# Autodesk Inventor assembly: roller
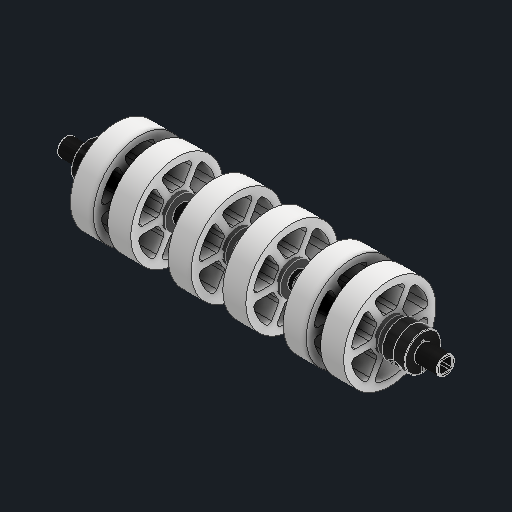
[picture p0: Inventor's stored thumbnail of the model, 512x512]
Saved by Autodesk Inventor 2024 (Build 280153000, 153)
## iProperties
Created: 2024-02-24
Part Number: roller
Document SubType Name: Assembly
Designer: Averey Ku
Author: Averey Ku
## Documents named in this file (8)
- D:\vex_robotics\hardware\cad\smolbot\intake\roller.iam
- D:\vex_robotics\hardware\cad\VEX-CAD-Inventor-1.41\Motion\Wheels\Flex Wheels\2.000 Flex Wheel\2.000 30A .500.ipt
- D:\vex_robotics\hardware\cad\VEX-CAD-Inventor-1.41\Motion\Wheels\Flex Wheels\VersaHex Adapters .125.ipt
- D:\vex_robotics\hardware\cad\VEX-CAD-Inventor-1.41\Motion\Shaft HS\HS Spacer\HSpacer .1250.ipt
- D:\vex_robotics\hardware\cad\VEX-CAD-Inventor-1.41\Motion\Shaft HS\HS Spacer\HSpacer .5000.ipt
- D:\vex_robotics\hardware\cad\VEX-CAD-Inventor-1.41\Motion\Shaft HS\HS Shaft Collar.ipt
- D:\vex_robotics\hardware\cad\VEX-CAD-Inventor-1.41\Motion\Wheels\Flex Wheels\2.000 Flex Wheel.ipt
- D:\vex_robotics\hardware\cad\VEX-CAD-Inventor-1.41\Motion\Shaft HS\HS Spacer.ipt
## Components (31 placed, 5 different names)
1. 2.000 30A .500:2 — Insert:20
2. VersaHex Adapters .125:3
3. VersaHex Adapters .125:4 — Insert:18, Insert:20
4. 2.000 30A .500:3 — Insert:21, Insert:22
5. VersaHex Adapters .125:5 — Insert:19, Insert:21
6. VersaHex Adapters .125:6 — Insert:22
7. 2.000 30A .500:4 — Insert:35
8. VersaHex Adapters .125:7 — Insert:23
9. VersaHex Adapters .125:8 — Insert:35, Insert:36
10. 2.000 30A .500:5 — Insert:33, Insert:34
11. VersaHex Adapters .125:9 — Insert:34
12. VersaHex Adapters .125:10 — Insert:31, Insert:33
13. 2.000 30A .500:6 — Insert:26, Insert:28
14. VersaHex Adapters .125:11 — Insert:28
15. VersaHex Adapters .125:12 — Insert:25, Insert:26
16. 2.000 30A .500:7 — Insert:27, Insert:30
17. VersaHex Adapters .125:13 — Insert:24, Insert:27, Insert:29
18. VersaHex Adapters .125:14 — Insert:30, Insert:32
19. HSpacer .5000:3 — Insert:36
20. HS Shaft Collar:1 — Insert:38
21. HSpacer .1250:6
22. HS Shaft Collar:2 — Insert:37
23. HSpacer .1250:7 — Insert:32
24. HSpacer .5000:8
25. HSpacer .1250:9 — Insert:31
26. HSpacer .5000:10
27. HSpacer .1250:11 — Insert:23
28. HSpacer .1250:14 — Insert:18, Insert:19
29. HSpacer .1250:15 — Insert:24, Insert:25, Insert:29
30. HSpacer .5000:16 — Insert:37
31. HSpacer .5000:17 — Insert:38
## Relationships (29: Insert 29)
- [Insert]: VersaHex Adapters .125:9 ↔ HSpacer .5000:3
- [Insert]: HS Shaft Collar:1 ↔ HSpacer .1250:6
- [Insert]: VersaHex Adapters .125:3 ↔ HSpacer .1250:6
- [Insert]: HS Shaft Collar:2 ↔ HSpacer .1250:7
- [Insert]: HSpacer .5000:8 ↔ HSpacer .1250:9
- [Insert]: HSpacer .5000:10 ↔ HSpacer .1250:11
- [Insert]: VersaHex Adapters .125:6 ↔ HSpacer .5000:10
- [Insert]: VersaHex Adapters .125:11 ↔ HSpacer .5000:8
- Insert:18: VersaHex Adapters .125:4 ↔ HSpacer .1250:14
- Insert:19: VersaHex Adapters .125:5 ↔ HSpacer .1250:14
- Insert:20: 2.000 30A .500:2 ↔ VersaHex Adapters .125:4
- Insert:21: 2.000 30A .500:3 ↔ VersaHex Adapters .125:5
- Insert:22: 2.000 30A .500:3 ↔ VersaHex Adapters .125:6
- Insert:23: VersaHex Adapters .125:7 ↔ HSpacer .1250:11
- Insert:24: VersaHex Adapters .125:13 ↔ HSpacer .1250:15
- Insert:25: VersaHex Adapters .125:12 ↔ HSpacer .1250:15
- Insert:26: 2.000 30A .500:6 ↔ VersaHex Adapters .125:12
- Insert:27: 2.000 30A .500:7 ↔ VersaHex Adapters .125:13
- Insert:28: 2.000 30A .500:6 ↔ VersaHex Adapters .125:11
- Insert:29: VersaHex Adapters .125:13 ↔ HSpacer .1250:15
- Insert:30: 2.000 30A .500:7 ↔ VersaHex Adapters .125:14
- Insert:31: VersaHex Adapters .125:10 ↔ HSpacer .1250:9
- Insert:32: VersaHex Adapters .125:14 ↔ HSpacer .1250:7
- Insert:33: 2.000 30A .500:5 ↔ VersaHex Adapters .125:10
- Insert:34: 2.000 30A .500:5 ↔ VersaHex Adapters .125:9
- Insert:35: 2.000 30A .500:4 ↔ VersaHex Adapters .125:8
- Insert:36: VersaHex Adapters .125:8 ↔ HSpacer .5000:3
- Insert:37: HS Shaft Collar:2 ↔ HSpacer .5000:16
- Insert:38: HS Shaft Collar:1 ↔ HSpacer .5000:17
## Named parameters: d7_d5 = 0 mm, d10_d9 = 0 mm
